# Autodesk Inventor assembly: RR
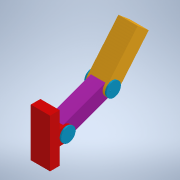
[picture p0: Inventor's stored thumbnail of the model, 180x180]
Saved by Autodesk Inventor 2021 (Build 250183000, 183)
## iProperties
Created: 2022-04-29
Part Number: RR
Document SubType Name: Assembly
Designer: Administrator
Title: Solution v2
Author: Administrator
## Documents named in this file (5)
- C:\Users\youss\OneDrive\Desktop\RR\RR.iam
- C:\Users\youss\OneDrive\Desktop\RR\Base v3.ipt
- C:\Users\youss\OneDrive\Desktop\RR\Motor v2.ipt
- C:\Users\youss\OneDrive\Desktop\RR\End v2.ipt
- C:\Users\youss\OneDrive\Desktop\RR\Middle v2.ipt
## Components (5 placed, 4 different names)
1. Base v3:1 — Rotational:1
2. Motor v2:1 — Rigid:1
3. Motor v2:2 — Rigid:2, Rotational:2
4. End v2:1 — Rigid:2
5. Middle v2:1 — Rigid:1, Rotational:1, Rotational:2
## Relationships (4: WeldJoint 2, RevoluteJoint 2)
- Rigid:1 [WeldJoint]: Motor v2:1 ↔ Middle v2:1
- Rotational:1 [RevoluteJoint]: Base v3:1 ↔ Middle v2:1
- Rigid:2 [WeldJoint]: Motor v2:2 ↔ End v2:1
- Rotational:2 [RevoluteJoint]: Motor v2:2 ↔ Middle v2:1
